# Autodesk Inventor assembly: FRP42-I110K_drivable
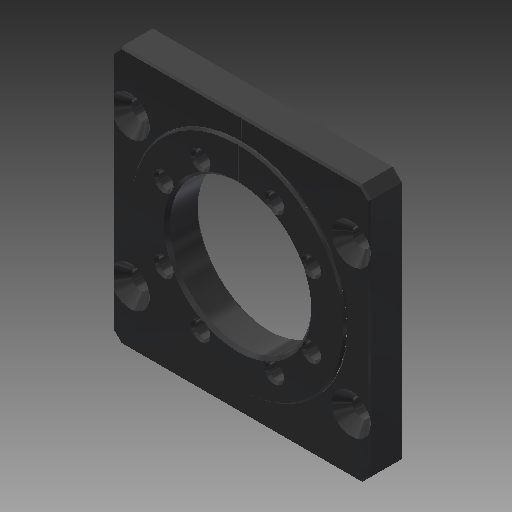
[picture p0: Inventor's stored thumbnail of the model, 512x512]
Saved by Autodesk Inventor 2023 (Build 270158000, 158)
## iProperties
Created: 2018-06-26
Part Number: FRP42-I110K_drivable
Material: 一般
Document SubType Name: Assembly
Designer: TAKEMORI
Mass: 18.6402 g
Surface Area: 54.6209 cm^2
Volume: 6.90379 cm^3
Density: 2.7 g/cm^3
Author: TAKEMORI
## Documents named in this file (3)
- C:\Users\michi\OneDrive - Kyoto University\lab\6_SHINOBI\FUHGA3\Design_Mechanism\Dynamixel\DynamixelPro_H42\FRP42-I110K_drivable.iam
- C:\Users\michi\OneDrive - Kyoto University\lab\6_SHINOBI\FUHGA3\Design_Mechanism\Dynamixel\DynamixelPro_H42\FRP42-I110K_without_hone.ipt
- C:\Users\michi\OneDrive - Kyoto University\lab\6_SHINOBI\FUHGA3\Design_Mechanism\Dynamixel\DynamixelPro_H42\FRP42-I110K_hone.ipt
## Components (2 placed, 2 different names)
1. FRP42-I110K_without_hone:1 — 挿入:1
2. FRP42-I110K_hone:1 — 挿入:1
## Relationships (1: Insert 1)
- 挿入:1 [Insert] (0.5 mm): FRP42-I110K_without_hone:1 ↔ FRP42-I110K_hone:1
